# Autodesk Inventor assembly: Reciprocating Saw
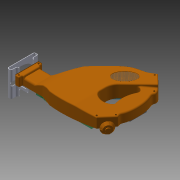
[picture p0: Inventor's stored thumbnail of the model, 180x180]
Saved by Autodesk Inventor 2015 (Build 190141000, 141)
## iProperties
Created: 2008-06-06
Part Number: Reciprocating Saw
Document SubType Name: Assembly
Designer: tangg
Mass: 711.371 g
Surface Area: 3987.93 cm^2
Volume: 242.811 cm^3
Density: 2.92973 g/cm^3
Author: tangg
## Documents named in this file (11)
- C:\Users\Aielloj\Downloads\inventor_2014_simulation\tutorial files\Dynamic Simulation 1 and 2\Reciprocating Saw.iam
- C:\Users\Aielloj\Downloads\inventor_2014_simulation\tutorial files\Dynamic Simulation 1 and 2\Saw layout.ipt
- C:\Users\Aielloj\Downloads\inventor_2014_simulation\tutorial files\Dynamic Simulation 1 and 2\Guide.ipt
- C:\Users\Aielloj\Downloads\inventor_2014_simulation\tutorial files\Dynamic Simulation 1 and 2\Motor housing.ipt
- C:\Users\Aielloj\Downloads\inventor_2014_simulation\tutorial files\Dynamic Simulation 1 and 2\Case.ipt
- C:\Users\Aielloj\Downloads\inventor_2014_simulation\tutorial files\Dynamic Simulation 1 and 2\Follower.ipt
- C:\Users\Aielloj\Downloads\inventor_2014_simulation\tutorial files\Dynamic Simulation 1 and 2\Fence.ipt
- C:\Users\Aielloj\Downloads\inventor_2014_simulation\tutorial files\Dynamic Simulation 1 and 2\Cam crank.iam
- C:\Users\Aielloj\Downloads\inventor_2014_simulation\tutorial files\Dynamic Simulation 1 and 2\Motor.iam
- C:\Users\Aielloj\Downloads\inventor_2014_simulation\tutorial files\Dynamic Simulation 1 and 2\Follower Roller.ipt
- C:\Users\Aielloj\Downloads\inventor_2014_simulation\tutorial files\Dynamic Simulation 1 and 2\SKFRLS 4 A-2ZANSI.ipt
## Components (11 placed, 10 different names)
1. Saw layout:1 — Flush:15, Mate:66, Mate:76, Mate:77
2. Case:1 — Flush:16, Mate:74, Flush:19, Flush:20
3. Fence:1 — Flush:16, Mate:74
4. Guide:1 — Flush:15, Mate:71, Mate:72
5. SKF Series RLS- with Two Shields RLS 4 A-2Z:1 — Flush:19
6. SKF Series RLS- with Two Shields RLS 4 A-2Z:2 — Flush:20
7. Motor housing:1 — Mate:66, Mate:73
8. Cam crank:1 [sub-assembly] — Mate:76, Mate:77
9. Motor:1 [sub-assembly] — Mate:73
10. Follower:1 — Mate:71, Mate:72, Mate:75, Flush:17
11. Follower Roller:1 — Mate:75, Flush:17
## Relationships (16: Mate 11, Flush 5)
- Flush:15: Saw layout:1 ↔ Guide:1
- Flush:16: Case:1 ↔ Fence:1
- Mate:66: Saw layout:1 ↔ Motor housing:1
- Mate:71: Guide:1 ↔ Follower:1
- Mate:72: Guide:1 ↔ Follower:1
- Mate:73: Motor housing:1 ↔ Motor:1
- Mate:74: Case:1 ↔ Fence:1
- Mate:75: Follower:1 ↔ Follower Roller:1
- Flush:17: Follower:1 ↔ Follower Roller:1
- Mate:76: Saw layout:1 ↔ Cam crank:1
- Mate:77: Saw layout:1 ↔ Cam crank:1
- [Mate]: Saw layout:1 ↔ Motor:1
- [Mate]: Case:1 ↔ SKF Series RLS- with Two Shields RLS 4 A-2Z:1
- Flush:19: Case:1 ↔ SKF Series RLS- with Two Shields RLS 4 A-2Z:1
- [Mate]: Case:1 ↔ SKF Series RLS- with Two Shields RLS 4 A-2Z:2
- Flush:20: Case:1 ↔ SKF Series RLS- with Two Shields RLS 4 A-2Z:2
